# Autodesk Inventor assembly: X-Gantry Assembly for 4040 V1
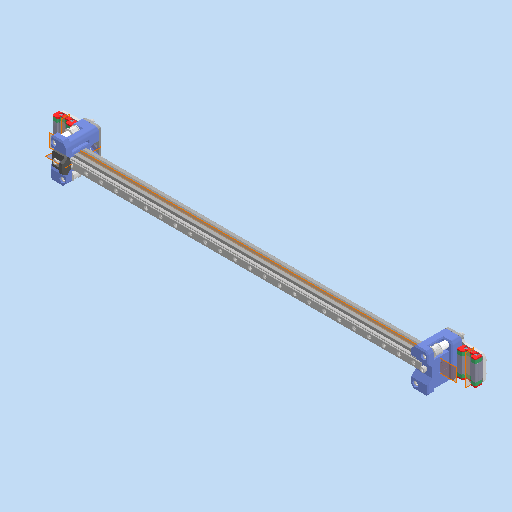
[picture p0: Inventor's stored thumbnail of the model, 512x512]
Saved by Autodesk Inventor 2023.2 (Build 272271000, 271)
## iProperties
Created: 2023-11-20
Part Number: X-Gantry Assembly for 4040 V1
Document SubType Name: Assembly
Designer: Nils Bade
Author: Nils Bade
## Documents named in this file (6)
- C:\Users\nilsb\Documents\Inventor\Projektarbeit-Bade\RatRig_Bade\X-Gantry Assembly for 4040 V1.iam
- X-Gantry Assembly for 4040 V1.iam
- C:\Users\nilsb\Documents\Inventor\Projektarbeit-Bade\RatRig_Standards\V-Slot 2020 - Black - 622mm v1.ipt
- C:\Users\nilsb\Documents\Inventor\Projektarbeit-Bade\RatRig_Standards\MGN12R 600mm 2020 Assembly v2.iam
- C:\Users\nilsb\Documents\Inventor\Projektarbeit-Bade\RatRig_Bade\X-Gantry Joiner Right Assembly.iam
- C:\Users\nilsb\Documents\Inventor\Projektarbeit-Bade\RatRig_Bade\X-Gantry Joiner Left Assembly.iam
## Components (4 placed, 4 different names)
1. V-Slot 2020 - Black - 622mm v1:1 — Passend:29, Fluchtend:31, Passend:30, Fluchtend:32, Fluchtend:33, Passend:31, Fluchtend:34, Passend:32, Passend:33
2. MGN12R 600mm 2020 Assembly v2:1 [sub-assembly] — Passend:29, Fluchtend:31, Passend:30
3. X-Gantry Joinder Right Assembly:1 [sub-assembly] — Fluchtend:34, Passend:32, Passend:33
4. X-Gantry Joiner Left Assembly:1 [sub-assembly] — Fluchtend:32, Fluchtend:33, Passend:31
## Relationships (9: Mate 5, Flush 4)
- Passend:29 [Mate]: V-Slot 2020 - Black - 622mm v1:1 ↔ MGN12R 600mm 2020 Assembly v2:1
- Fluchtend:31 [Flush]: V-Slot 2020 - Black - 622mm v1:1 ↔ MGN12R 600mm 2020 Assembly v2:1
- Passend:30 [Mate]: V-Slot 2020 - Black - 622mm v1:1 ↔ MGN12R 600mm 2020 Assembly v2:1
- Fluchtend:32 [Flush]: V-Slot 2020 - Black - 622mm v1:1 ↔ X-Gantry Joiner Left Assembly:1
- Fluchtend:33 [Flush]: V-Slot 2020 - Black - 622mm v1:1 ↔ X-Gantry Joiner Left Assembly:1
- Passend:31 [Mate]: V-Slot 2020 - Black - 622mm v1:1 ↔ X-Gantry Joiner Left Assembly:1
- Fluchtend:34 [Flush]: V-Slot 2020 - Black - 622mm v1:1 ↔ X-Gantry Joinder Right Assembly:1
- Passend:32 [Mate]: V-Slot 2020 - Black - 622mm v1:1 ↔ X-Gantry Joinder Right Assembly:1
- Passend:33 [Mate]: V-Slot 2020 - Black - 622mm v1:1 ↔ X-Gantry Joinder Right Assembly:1
